# Autodesk Inventor assembly: Left_Arm
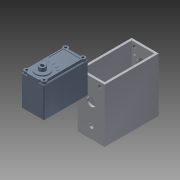
[picture p0: Inventor's stored thumbnail of the model, 180x180]
Saved by Autodesk Inventor 2013 (Build 170138000, 138)
## iProperties
Created: 2014-05-07
Part Number: Left_Arm
Document SubType Name: Assembly
Designer: andou
Author: andou
## Documents named in this file (3)
- C:\Users\andou\Documents\Inventor\RoboticsProject\project_4\Robot\Left_Arm.iam
- C:\Users\andou\Documents\Inventor\RoboticsProject\project_4\Robot\Serial_Case.ipt
- C:\Users\andou\Documents\Inventor\RoboticsProject\project_4\Robot\KRS-2542HV.ipt
## Components (2 placed, 2 different names)
1. Serial_Case:1 — メイト:1
2. KRS-2542HV:1 — メイト:1
## Relationships (1: Mate 1)
- メイト:1 [Mate]: Serial_Case:1 ↔ KRS-2542HV:1
